# Autodesk Inventor assembly: Motor Mount with Motor
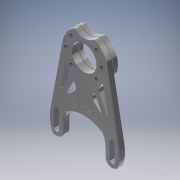
[picture p0: Inventor's stored thumbnail of the model, 180x180]
Saved by Autodesk Inventor 2019.4 (Build 234330000, 330)
## iProperties
Created: 2019-03-01
Part Number: Motor Mount with Motor
Document SubType Name: Assembly
Designer: Petar
Mass: 37.7633 g
Surface Area: 102.459 cm^2
Volume: 12.7696 cm^3
Density: 2.95729 g/cm^3
Author: Petar
## Documents named in this file (3)
- D:\OMG\E-Board\CAD\Inventor\Mechanical Components\Assemblies\Motor Mount - 225.iam
- D:\OMG\E-Board\CAD\Inventor\Mechanical Components\Motor Mount\Ring Mount\Mount Ring - ALUMINIUM.ipt
- D:\OMG\E-Board\CAD\Inventor\Mechanical Components\Motor Mount\Holder Mount\Motor Holder v3 - 225 - ALUMINIUM.ipt
## Components (2 placed, 2 different names)
1. Motor Holder v3 - 225 - ALUMINIUM:1 — Rigid:2
2. Mount Ring - ALUMINIUM:1 — Rigid:2
## Relationships (1: WeldJoint 1)
- Rigid:2 [WeldJoint]: Motor Holder v3 - 225 - ALUMINIUM:1 ↔ Mount Ring - ALUMINIUM:1
